# Autodesk Inventor assembly: Hexapod
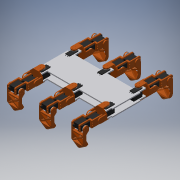
[picture p0: Inventor's stored thumbnail of the model, 180x180]
Saved by Autodesk Inventor 2017 (Build 210142000, 142)
## iProperties
Created: 2017-01-26
Part Number: Hexapod
Document SubType Name: Assembly
Designer: Alexander Miller
Author: Alexander Miller
## Documents named in this file (3)
- D:\Daten\Documents\Git\Hexapod\3DParts\HexPi_v2\Hexapod.iam
- D:\Daten\Documents\Git\Hexapod\3DParts\HexPi_v2\Body.iam
- D:\Daten\Documents\Git\Hexapod\3DParts\HexPi_v2\Leg.iam
## Components (7 placed, 2 different names)
1. Body:1 [sub-assembly] — Rigid:1, Rigid:2, Rigid:3, Rigid:4, Rigid:5, Rigid:6
2. Leg:1 [sub-assembly] — Rigid:1
3. Leg:2 [sub-assembly] — Rigid:2
4. Leg:3 [sub-assembly] — Rigid:3
5. Leg:4 [sub-assembly] — Rigid:4
6. Leg:5 [sub-assembly] — Rigid:5
7. Leg:6 [sub-assembly] — Rigid:6
## Relationships (6: WeldJoint 6)
- Rigid:1 [WeldJoint]: Body:1 ↔ Leg:1
- Rigid:2 [WeldJoint]: Body:1 ↔ Leg:2
- Rigid:3 [WeldJoint]: Body:1 ↔ Leg:3
- Rigid:4 [WeldJoint]: Body:1 ↔ Leg:4
- Rigid:5 [WeldJoint]: Body:1 ↔ Leg:5
- Rigid:6 [WeldJoint]: Body:1 ↔ Leg:6
